# Autodesk Inventor assembly: Assembly1
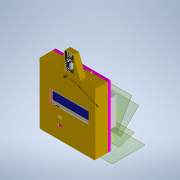
[picture p0: Inventor's stored thumbnail of the model, 180x180]
Saved by Autodesk Inventor 2021 (Build 250183000, 183)
## iProperties
Created: 2021-07-02
Part Number: Assembly1
Document SubType Name: Assembly
Designer: Admin
Author: Admin
## Documents named in this file (12)
- C:\Users\Admin\Documents\UVG\Ultimo Semestre\Diseno e Innovacion 2\Disenos 3D\Assembly1.iam
- C:\Users\Admin\Documents\UVG\Ultimo Semestre\Diseno e Innovacion 2\Disenos 3D\LCDPCF8574.iam
- C:\Users\Admin\Documents\UVG\Ultimo Semestre\Diseno e Innovacion 2\Disenos 3D\lcd-16x2-5.snapshot.1\LCD16X2\LCD 16X2.ipt
- C:\Users\Admin\Documents\UVG\Ultimo Semestre\Diseno e Innovacion 2\Disenos 3D\nodemcu-esp8266-esp-12e-1.snapshot.1\nodemcu ESP8266 ESP-12E.ipt
- C:\Users\Admin\Documents\UVG\Ultimo Semestre\Diseno e Innovacion 2\Disenos 3D\Base de CObre.ipt
- C:\Users\Admin\Documents\UVG\Ultimo Semestre\Diseno e Innovacion 2\Disenos 3D\pin-header-female-double-2-54mm-different-pin-numbers-1.snapshot.2\16-Pin Header - Female - 2.54mm.ipt
- C:\Users\Admin\Documents\UVG\Ultimo Semestre\Diseno e Innovacion 2\Disenos 3D\pin-header-female-double-2-54mm-different-pin-numbers-1.snapshot.2\15-Pin Header - Female - 2.54mm.ipt
- C:\Users\Admin\Documents\UVG\Ultimo Semestre\Diseno e Innovacion 2\Disenos 3D\pin-header-female-double-2-54mm-different-pin-numbers-1.snapshot.2\8-Pin Header - Female - Double - 2.54mm.ipt
- C:\Users\Admin\Documents\UVG\Ultimo Semestre\Diseno e Innovacion 2\Disenos 3D\Cubierta parte 1.ipt
- C:\Users\Admin\Documents\UVG\Ultimo Semestre\Diseno e Innovacion 2\Disenos 3D\Cubierta SUperior.ipt
- C:\Users\Admin\Documents\UVG\Ultimo Semestre\Diseno e Innovacion 2\Disenos 3D\wireless-radio-transmitter-and-receiver-nrf24l01-1.snapshot.5\Wireless Radio Transmitter and Receiver nRF24L01.ipt
- C:\Users\Admin\Documents\UVG\Ultimo Semestre\Diseno e Innovacion 2\Disenos 3D\Part17.ipt
## Components (13 placed, 11 different names)
1. LCDPCF8574:1 [sub-assembly] — Mate:6, Mate:7, Mate:8
2. LCD 16X2:1 — Rigid:1
3. nodemcu ESP8266 ESP-12E:1 — Rigid:2
4. Base de CObre:1 — Mate:4, Flush:3, Flush:4, Mate:5, Flush:5, Flush:6, Flush:7, Flush:8, Mate:9, Mate:11, Mate:12, Flush:10, Flush:11, Flush:12
5. 16-Pin Header - Female - 2.54mm:1 — Mate:4, Flush:3, Flush:4, Rigid:1
6. 16-Pin Header - Female - 2.54mm:2 — Mate:5, Flush:5, Flush:6, Mate:6, Mate:7, Mate:8
7. 15-Pin Header - Female - 2.54mm:1 — Mate:10, Flush:9, Mate:11
8. 15-Pin Header - Female - 2.54mm:2 — Flush:7, Flush:8, Mate:9, Mate:10, Flush:9, Rigid:2
9. 8-Pin Header - Female - Double - 2.54mm:1 — Mate:12, Flush:10, Flush:11
10. Cubierta parte 1:1 — Flush:12, Mate:13, Flush:14
11. Cubierta SUperior:1 — Mate:13, Mate:14, Mate:15, Flush:13
12. Wireless Radio Transmitter and Receiver nRF24L01:1 — Mate:14, Mate:15, Flush:13
13. Part17:1 — Flush:14
## Relationships (26: Mate 12, Flush 12, WeldJoint 2)
- Mate:4: Base de CObre:1 ↔ 16-Pin Header - Female - 2.54mm:1
- Flush:3 (14.2 mm): Base de CObre:1 ↔ 16-Pin Header - Female - 2.54mm:1
- Flush:4 (70 mm): Base de CObre:1 ↔ 16-Pin Header - Female - 2.54mm:1
- Rigid:1 [WeldJoint]: LCD 16X2:1 ↔ 16-Pin Header - Female - 2.54mm:1
- Mate:5: Base de CObre:1 ↔ 16-Pin Header - Female - 2.54mm:2
- Flush:5 (21.5 mm): Base de CObre:1 ↔ 16-Pin Header - Female - 2.54mm:2
- Flush:6 (18.3 mm): Base de CObre:1 ↔ 16-Pin Header - Female - 2.54mm:2
- Mate:6: LCDPCF8574:1 ↔ 16-Pin Header - Female - 2.54mm:2
- Mate:7: LCDPCF8574:1 ↔ 16-Pin Header - Female - 2.54mm:2
- Mate:8: LCDPCF8574:1 ↔ 16-Pin Header - Female - 2.54mm:2
- Flush:7 (10.5 mm): Base de CObre:1 ↔ 15-Pin Header - Female - 2.54mm:2
- Flush:8 (33 mm): Base de CObre:1 ↔ 15-Pin Header - Female - 2.54mm:2
- Mate:9: Base de CObre:1 ↔ 15-Pin Header - Female - 2.54mm:2
- Mate:10 (20 mm): 15-Pin Header - Female - 2.54mm:1 ↔ 15-Pin Header - Female - 2.54mm:2
- Flush:9: 15-Pin Header - Female - 2.54mm:1 ↔ 15-Pin Header - Female - 2.54mm:2
- Mate:11: Base de CObre:1 ↔ 15-Pin Header - Female - 2.54mm:1
- Rigid:2 [WeldJoint]: nodemcu ESP8266 ESP-12E:1 ↔ 15-Pin Header - Female - 2.54mm:2
- Mate:12: Base de CObre:1 ↔ 8-Pin Header - Female - Double - 2.54mm:1
- Flush:10 (4.8 mm): Base de CObre:1 ↔ 8-Pin Header - Female - Double - 2.54mm:1
- Flush:11 (16.25 mm): Base de CObre:1 ↔ 8-Pin Header - Female - Double - 2.54mm:1
- Flush:12: Base de CObre:1 ↔ Cubierta parte 1:1
- Mate:13: Cubierta parte 1:1 ↔ Cubierta SUperior:1
- Mate:14: Cubierta SUperior:1 ↔ Wireless Radio Transmitter and Receiver nRF24L01:1
- Mate:15: Cubierta SUperior:1 ↔ Wireless Radio Transmitter and Receiver nRF24L01:1
- Flush:13: Cubierta SUperior:1 ↔ Wireless Radio Transmitter and Receiver nRF24L01:1
- Flush:14: Cubierta parte 1:1 ↔ Part17:1
